# Autodesk Inventor assembly: RobotV3
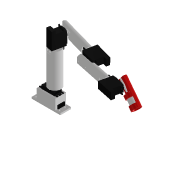
[picture p0: Inventor's stored thumbnail of the model, 180x180]
Saved by Autodesk Inventor 2022 (Build 260153000, 153)
## iProperties
Created: 2022-03-09
Part Number: RobotV3
Document SubType Name: Assembly
Designer: piers
Author: piers
## Documents named in this file (8)
- C:\Users\piers\OneDrive\Documents\Inventor\Robotics Project\RobotV3.iam
- C:\Users\piers\OneDrive\Documents\Inventor\Robotics Project\magnet assembly.iam
- C:\Users\piers\OneDrive\Documents\Inventor\Robotics Project\Motorv2.ipt
- C:\Users\piers\OneDrive\Documents\Inventor\Robotics Project\180Horn.ipt
- C:\Users\piers\OneDrive\Documents\Inventor\Robotics Project\90Horn.ipt
- C:\Users\piers\OneDrive\Documents\Inventor\Robotics Project\base.ipt
- C:\Users\piers\OneDrive\Documents\Inventor\Robotics Project\link1.ipt
- C:\Users\piers\OneDrive\Documents\Inventor\Robotics Project\link2.ipt
## Components (13 placed, 7 different names)
1. magnet assembly:1 [sub-assembly] — Mate:29, Mate:34, Mate:35
2. Motorv2:1 — Mate:18, Mate:19, Mate:20, Mate:21, Flush:3
3. Motorv2:2 — Mate:10, Mate:11, Mate:12, Mate:13, Flush:2
4. Motorv2:4 — Mate:1, Mate:2, Mate:6, Mate:7, Flush:1
5. 180Horn:1 — Mate:21, Flush:3, Mate:22, Mate:32, Mate:33
6. 180Horn:2 — Mate:28, Flush:4, Mate:29, Mate:34, Mate:35
7. 180Horn:4 — Mate:13, Flush:2, Mate:15, Mate:30, Mate:31
8. 90Horn:1 — Mate:7, Flush:1, Mate:8, Mate:9
9. base:1 — Mate:1, Mate:2, Mate:3, Mate:4, Mate:5, Mate:6
10. link1:1 — Mate:8, Mate:9, Mate:10, Mate:11, Mate:12
11. link2:1 — Mate:15, Mate:18, Mate:19, Mate:20, Mate:30, Mate:31
12. link2:2 — Mate:22, Mate:25, Mate:26, Mate:27, Mate:32, Mate:33
13. Motorv2:5 — Mate:25, Mate:26, Mate:27, Mate:28, Flush:4
## Relationships (34: Mate 30, Flush 4)
- Mate:1: Motorv2:4 ↔ base:1
- Mate:2 (1 mm): Motorv2:4 ↔ base:1
- Mate:3: base:1
- Mate:4: base:1
- Mate:5: base:1
- Mate:6 (1 mm): Motorv2:4 ↔ base:1
- Mate:7: Motorv2:4 ↔ 90Horn:1
- Flush:1: Motorv2:4 ↔ 90Horn:1
- Mate:8: 90Horn:1 ↔ link1:1
- Mate:9: 90Horn:1 ↔ link1:1
- Mate:10: Motorv2:2 ↔ link1:1
- Mate:11: Motorv2:2 ↔ link1:1
- Mate:12: Motorv2:2 ↔ link1:1
- Mate:13: Motorv2:2 ↔ 180Horn:4
- Flush:2: Motorv2:2 ↔ 180Horn:4
- Mate:15: 180Horn:4 ↔ link2:1
- Mate:18: Motorv2:1 ↔ link2:1
- Mate:19: Motorv2:1 ↔ link2:1
- Mate:20: Motorv2:1 ↔ link2:1
- Mate:21: Motorv2:1 ↔ 180Horn:1
- Flush:3: Motorv2:1 ↔ 180Horn:1
- Mate:22: 180Horn:1 ↔ link2:2
- Mate:25: link2:2 ↔ Motorv2:5
- Mate:26: link2:2 ↔ Motorv2:5
- Mate:27: link2:2 ↔ Motorv2:5
- Mate:28: 180Horn:2 ↔ Motorv2:5
- Flush:4: 180Horn:2 ↔ Motorv2:5
- Mate:29: magnet assembly:1 ↔ 180Horn:2
- Mate:30: 180Horn:4 ↔ link2:1
- Mate:31: 180Horn:4 ↔ link2:1
- Mate:32: 180Horn:1 ↔ link2:2
- Mate:33: 180Horn:1 ↔ link2:2
- Mate:34: magnet assembly:1 ↔ 180Horn:2
- Mate:35: magnet assembly:1 ↔ 180Horn:2
